# Autodesk Inventor assembly: Rubix
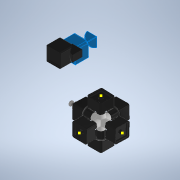
[picture p0: Inventor's stored thumbnail of the model, 180x180]
Saved by Autodesk Inventor 2020 (Build 240168000, 168)
## iProperties
Created: 2019-10-21
Part Number: Rubix
Document SubType Name: Assembly
Designer: eduso287260
Author: eduso287260
## Documents named in this file (9)
- C:\Users\Paul Koch\Dropbox\projecten paul\School\inventor files Paul\Les 6\Rubix.iam
- C:\Users\Paul Koch\Dropbox\projecten paul\School\inventor files Paul\Les 6\core.ipt
- C:\Users\Paul Koch\Dropbox\projecten paul\School\inventor files Paul\Les 6\corner-piece.ipt
- C:\Users\Paul Koch\Dropbox\projecten paul\School\inventor files Paul\Les 6\middle-piece.ipt
- C:\Users\Paul Koch\Dropbox\projecten paul\School\inventor files Paul\Les 6\middle-centre-piece.ipt
- C:\Users\Paul Koch\Dropbox\projecten paul\School\inventor files Paul\Les 6\Ring.ipt
- C:\Users\Paul Koch\Dropbox\projecten paul\School\inventor files Paul\Les 6\Spring.ipt
- C:\Users\Paul Koch\Documents\Inventor\Content Center Files\R2020\en-US\AS 1427(01)\AS 1427 - M3 x 20(3).ipt
- C:\Users\Paul Koch\Dropbox\projecten paul\School\inventor files Paul\Les 6\cube-inlay-red.ipt
## Components (13 placed, 8 different names)
1. core:1 — Mate:1, Mate:2, Mate:3, Mate:4, Mate:5, Mate:6, Mate:7, Mate:8, Mate:9, Mate:10, Mate:11, Mate:12
2. corner-piece:1
3. middle-piece:1 — Transitional:1, Transitional:2, Flush:1
4. middle-centre-piece:1 — Mate:3, Mate:4
5. middle-centre-piece:2 — Mate:9, Mate:10
6. middle-centre-piece:3 — Mate:11, Mate:12
7. middle-centre-piece:4 — Mate:1, Mate:2, Mate:13, Mate:14, Mate:15
8. middle-centre-piece:5 — Mate:5, Mate:6
9. middle-centre-piece:6 — Mate:7, Mate:8
10. Ring:1 — Mate:13
11. Spring:1 — Mate:14
12. AS 1427 - Metric M3 x 20:1 — Mate:15
13. cube-inlay-red:1 — Transitional:1, Transitional:2, Flush:1
## Relationships (18: Mate 15, Transitional 2, Flush 1)
- Mate:1: core:1 ↔ middle-centre-piece:4
- Mate:2: core:1 ↔ middle-centre-piece:4
- Mate:3: core:1 ↔ middle-centre-piece:1
- Mate:4: core:1 ↔ middle-centre-piece:1
- Mate:5: core:1 ↔ middle-centre-piece:5
- Mate:6: core:1 ↔ middle-centre-piece:5
- Mate:7: core:1 ↔ middle-centre-piece:6
- Mate:8: core:1 ↔ middle-centre-piece:6
- Mate:9: core:1 ↔ middle-centre-piece:2
- Mate:10: core:1 ↔ middle-centre-piece:2
- Mate:11: core:1 ↔ middle-centre-piece:3
- Mate:12: core:1 ↔ middle-centre-piece:3
- Mate:13: middle-centre-piece:4 ↔ Ring:1
- Mate:14: middle-centre-piece:4 ↔ Spring:1
- Mate:15: middle-centre-piece:4 ↔ AS 1427 - Metric M3 x 20:1
- Transitional:1: middle-piece:1 ↔ cube-inlay-red:1
- Transitional:2: middle-piece:1 ↔ cube-inlay-red:1
- Flush:1: middle-piece:1 ↔ cube-inlay-red:1
